# Autodesk Inventor assembly: Assembly
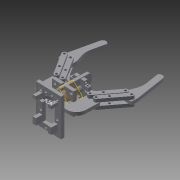
[picture p0: Inventor's stored thumbnail of the model, 180x180]
Saved by Autodesk Inventor 2015 (Build 190159000, 159)
## iProperties
Created: 2016-10-14
Part Number: Assembly
Document SubType Name: Assembly
Designer: Bardo91
Author: Bardo91
## Documents named in this file (10)
- C:\Users\Bardo91\Dropbox\GRVC\cadHexacopter\RobotArm\gripper\Assembly.iam
- C:\Users\Bardo91\Dropbox\GRVC\cadHexacopter\RobotArm\gripper\holdBar.ipt
- C:\Users\Bardo91\Dropbox\GRVC\cadHexacopter\RobotArm\gripper\bar.ipt
- C:\Users\Bardo91\Dropbox\GRVC\cadHexacopter\RobotArm\gripper\gripper.ipt
- C:\Users\Bardo91\Dropbox\GRVC\cadHexacopter\RobotArm\gripper\barMini.ipt
- C:\Users\Bardo91\Dropbox\GRVC\cadHexacopter\RobotArm\gripper\block.ipt
- C:\Users\Bardo91\Dropbox\GRVC\cadHexacopter\RobotArm\gripper\servorPlace.ipt
- C:\Users\Bardo91\Dropbox\GRVC\cadHexacopter\RobotArm\gripper\crossCenterBlock.ipt
- C:\Users\Bardo91\Dropbox\GRVC\cadHexacopter\RobotArm\gripper\crossCenterMiniBlock.ipt
- C:\Users\Bardo91\Dropbox\GRVC\cadHexacopter\RobotArm\gripper\screwServoBlock.ipt
## Components (20 placed, 9 different names)
1. holdBar:1 — Mate:1, Mate:2, Mate:3, Mate:4, Mate:5, Mate:6, Mate:7, Mate:8, Mate:48, Mate:49
2. bar:1 — Mate:3, Mate:4, Mate:11, Mate:13, Mate:14, Mate:15
3. bar:2 — Mate:5, Mate:7, Mate:10
4. bar:3 — Mate:6, Mate:8, Mate:12
5. bar:4 — Mate:1, Mate:2, Mate:9
6. gripper:1 — Mate:9, Mate:10, Mate:11, Mate:12, Mate:13
7. barMini:1 — Mate:14, Mate:15, Mate:46
8. bar:5 — Mate:25, Mate:26, Mate:32
9. bar:6 — Mate:24, Mate:29, Mate:34
10. bar:7 — Mate:23, Mate:27, Mate:30, Mate:31, Mate:38, Mate:39
11. bar:8 — Mate:22, Mate:28, Mate:33
12. holdBar:2 — Mate:30, Mate:31, Mate:32, Mate:33, Mate:34, Mate:41, Mate:42, Mate:43
13. gripper:2 — Mate:22, Mate:23, Mate:24, Mate:25, Mate:26, Mate:27, Mate:28, Mate:29
14. barMini:2 — Mate:38, Mate:39, Mate:44, Mate:45
15. block:1
16. block:2
17. servorPlace:1 — Mate:50
18. crossCenterBlock:1 — Mate:41, Mate:42, Mate:43, Mate:48, Mate:49
19. crossCenterMiniBlock:1 — Mate:44, Mate:45, Mate:46, Mate:51
20. screwServoBlock:1 — Mate:50, Mate:51
## Relationships (40: Mate 40)
- Mate:1: holdBar:1 ↔ bar:4
- Mate:2: holdBar:1 ↔ bar:4
- Mate:3: holdBar:1 ↔ bar:1
- Mate:4: holdBar:1 ↔ bar:1
- Mate:5: holdBar:1 ↔ bar:2
- Mate:6: holdBar:1 ↔ bar:3
- Mate:7: holdBar:1 ↔ bar:2
- Mate:8: holdBar:1 ↔ bar:3
- Mate:9: bar:4 ↔ gripper:1
- Mate:10: bar:2 ↔ gripper:1
- Mate:11: bar:1 ↔ gripper:1
- Mate:12: bar:3 ↔ gripper:1
- Mate:13: bar:1 ↔ gripper:1
- Mate:14: bar:1 ↔ barMini:1
- Mate:15: bar:1 ↔ barMini:1
- Mate:22: bar:8 ↔ gripper:2
- Mate:23: bar:7 ↔ gripper:2
- Mate:24: bar:6 ↔ gripper:2
- Mate:25: bar:5 ↔ gripper:2
- Mate:26: bar:5 ↔ gripper:2
- Mate:27: bar:7 ↔ gripper:2
- Mate:28: bar:8 ↔ gripper:2
- Mate:29: bar:6 ↔ gripper:2
- Mate:30: bar:7 ↔ holdBar:2
- Mate:31: bar:7 ↔ holdBar:2
- Mate:32: bar:5 ↔ holdBar:2
- Mate:33: bar:8 ↔ holdBar:2
- Mate:34: bar:6 ↔ holdBar:2
- Mate:38: bar:7 ↔ barMini:2
- Mate:39: bar:7 ↔ barMini:2
- Mate:41: holdBar:2 ↔ crossCenterBlock:1
- Mate:42: holdBar:2 ↔ crossCenterBlock:1
- Mate:43: holdBar:2 ↔ crossCenterBlock:1
- Mate:44: barMini:2 ↔ crossCenterMiniBlock:1
- Mate:45: barMini:2 ↔ crossCenterMiniBlock:1
- Mate:46: barMini:1 ↔ crossCenterMiniBlock:1
- Mate:48: holdBar:1 ↔ crossCenterBlock:1
- Mate:49: holdBar:1 ↔ crossCenterBlock:1
- Mate:50 (10 mm): servorPlace:1 ↔ screwServoBlock:1
- Mate:51: crossCenterMiniBlock:1 ↔ screwServoBlock:1
